# Autodesk Inventor assembly: endplate_ver2
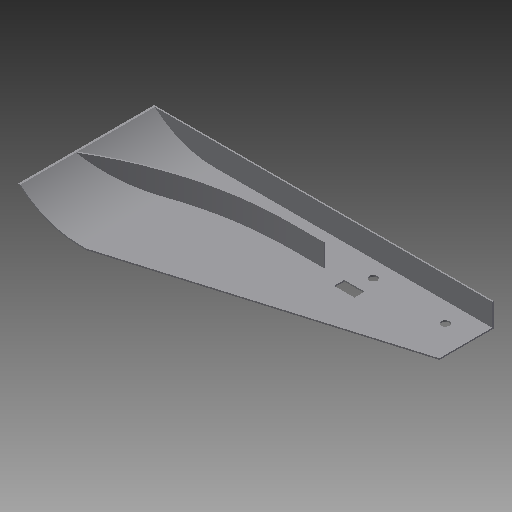
[picture p0: Inventor's stored thumbnail of the model, 512x512]
Saved by Autodesk Inventor 2018 (Build 220112000, 112)
## iProperties
Created: 2018-05-29
Part Number: endplate_ver2
Material: 一般
Document SubType Name: Assembly
Designer: ku_sk
Author: ku_sk
## Documents named in this file (3)
- D:\Users\ku_sk\Documents\Inventor\Aero\KS-15\Fr.wing\parts\endplate\ver.2\endplate_ver2.iam
- D:\Users\ku_sk\Documents\Inventor\Aero\KS-15\Fr.wing\parts\endplate\ver.2\parts\Part1.ipt
- D:\Users\ku_sk\Documents\Inventor\Aero\KS-15\Fr.wing\parts\endplate\ver.2\parts\Part2.ipt
## Components (2 placed, 2 different names)
1. Part1:1 — メイト:1, メイト:2, メイト:3, メイト:4, メイト:5, メイト:6
2. Part2:1 — メイト:1, メイト:2, メイト:3
## Relationships (6: Mate 6)
- メイト:1 [Mate]: Part1:1 ↔ Part2:1
- メイト:2 [Mate]: Part1:1 ↔ Part2:1
- メイト:3 [Mate]: Part1:1 ↔ Part2:1
- メイト:4 [Mate]: Part1:1
- メイト:5 [Mate]: Part1:1
- メイト:6 [Mate]: Part1:1
